# Autodesk Inventor assembly: Stock Dicoeasy Assembly-just x axis and platform
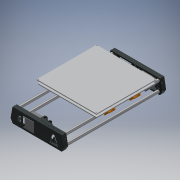
[picture p0: Inventor's stored thumbnail of the model, 180x180]
Saved by Autodesk Inventor 2017 (Build 210142000, 142)
## iProperties
Created: 2017-03-10
Part Number: Stock Dicoeasy Assembly-just x axis and platform
Document SubType Name: Assembly
Designer: gilef
Author: gilef
## Documents named in this file (14)
- C:\Users\gilef\Documents\Inventor\DiscoEasy200\Stock Dicoeasy Assembly-just x axis and platform.iam
- C:\Users\gilef\Documents\Inventor\DiscoEasy200\Original Plate Mount.ipt
- C:\Users\gilef\Documents\Inventor\DiscoEasy200\Original Rear Left Plate Mount.ipt
- C:\Users\gilef\Documents\Inventor\DiscoEasy200\Original Rear Right Plate Mount.ipt
- C:\Users\gilef\Documents\Inventor\DiscoEasy200\Converted LM8UU Linear Bearing.ipt
- C:\Users\gilef\Documents\Inventor\DiscoEasy200\Stock Build Plate.ipt
- C:\Users\gilef\Documents\Inventor\Content Center Files\R2017\en-US\AS 1427(07)\AS 1427 - M3 x 10(6) II.ipt
- C:\Users\gilef\Documents\Inventor\Content Center Files\R2017\en-US\ANSI B18.16.3M(2)\ANSI B18.16.3M - Property Class 5 and 10 - Metric M3 x 0.5 Metal Type.ipt
- C:\Users\gilef\Documents\Inventor\DiscoEasy200\Stock Front Plate.ipt
- C:\Users\gilef\Documents\Inventor\DiscoEasy200\Stock Back Plate.ipt
- C:\Users\gilef\Documents\Inventor\DiscoEasy200\Long Metal Rod.ipt
- C:\Users\gilef\Documents\Inventor\DiscoEasy200\XY Stepper Motor.ipt
- C:\Users\gilef\Documents\Inventor\DiscoEasy200\Heated Build Plate.ipt
- C:\Users\gilef\Documents\Inventor\DiscoEasy200\Plate Adapter.ipt
## Components (26 placed, 13 different names)
1. Original Plate Mount:1 — Flush:2, Mate:1, Flush:3, Mate:2, Mate:7, Mate:8, Mate:9, Mate:10, Mate:11, Insert:7, Angle:3, Insert:10, Angle:4
2. Original Rear Right Plate Mount:1 — Flush:2, Mate:1, Mate:3, Mate:4, Flush:4, Insert:9, Angle:1
3. Original Rear Left Plate Mount:1 — Flush:3, Mate:2, Mate:5, Mate:6, Flush:4, Insert:1, Insert:6, Angle:2
4. Converted LM8UU Linear Bearing:1 — Mate:7, Mate:8, Mate:15
5. Converted LM8UU Linear Bearing:2 — Mate:3, Mate:4, Mate:12
6. Converted LM8UU Linear Bearing:3 — Mate:9, Mate:10, Mate:14
7. Converted LM8UU Linear Bearing:4 — Mate:5, Mate:6, Mate:13
8. Stock Build Plate:1 — Insert:1, Mate:11, Insert:2, Insert:3, Insert:4, Insert:5, Mate:82, Angle:9, Flush:7, Flush:8, Mate:83, Mate:84, Mate:85
9. AS 1427 Z - Metric M3 x 10:1 — Insert:2
10. AS 1427 Z - Metric M3 x 10:2 — Insert:3
11. AS 1427 Z - Metric M3 x 10:3 — Insert:4
12. AS 1427 Z - Metric M3 x 10:4 — Insert:5
13. Prevailing Torque Type Hex Nut - Steel Metric Property Class 5 and 10 - Metric M3 x 0.5 Metal Type:1 — Insert:10, Angle:4
14. Prevailing Torque Type Hex Nut - Steel Metric Property Class 5 and 10 - Metric M3 x 0.5 Metal Type:2 — Insert:9, Angle:1
15. Prevailing Torque Type Hex Nut - Steel Metric Property Class 5 and 10 - Metric M3 x 0.5 Metal Type:3 — Insert:7, Angle:3
16. Prevailing Torque Type Hex Nut - Steel Metric Property Class 5 and 10 - Metric M3 x 0.5 Metal Type:4 — Insert:6, Angle:2
17. Stock Front Plate:1 — Mate:14, Mate:15, Insert:14, Insert:15, Insert:16, Insert:17, Mate:81, Angle:8, Flush:5, Flush:6
18. Stock Back Plate:1 — Mate:12, Mate:13, Insert:13, Mate:80, Tangent:1, Angle:7, Tangent:2
19. Long Metal Rod:1 — Insert:16
20. Long Metal Rod:2 — Insert:15
21. Long Metal Rod:3 — Insert:17
22. Long Metal Rod:4 — Insert:13, Insert:14
23. XY Stepper Motor:2 — Mate:80, Tangent:1, Angle:7, Tangent:2
24. XY Stepper Motor:3 — Mate:81, Angle:8, Flush:5, Flush:6
25. Heated Build Plate:1 — Mate:82, Angle:9, Flush:7, Flush:8
26. Plate Adapter:1 — Mate:83, Mate:84, Mate:85
## Relationships (51: Mate 21, Insert 14, Flush 7, Angle 7, Tangent 2)
- Flush:2: Original Plate Mount:1 ↔ Original Rear Right Plate Mount:1
- Mate:1: Original Plate Mount:1 ↔ Original Rear Right Plate Mount:1
- Flush:3: Original Plate Mount:1 ↔ Original Rear Left Plate Mount:1
- Mate:2: Original Plate Mount:1 ↔ Original Rear Left Plate Mount:1
- Mate:3: Original Rear Right Plate Mount:1 ↔ Converted LM8UU Linear Bearing:2
- Mate:4: Original Rear Right Plate Mount:1 ↔ Converted LM8UU Linear Bearing:2
- Mate:5: Original Rear Left Plate Mount:1 ↔ Converted LM8UU Linear Bearing:4
- Mate:6: Original Rear Left Plate Mount:1 ↔ Converted LM8UU Linear Bearing:4
- Mate:7: Original Plate Mount:1 ↔ Converted LM8UU Linear Bearing:1
- Mate:8: Original Plate Mount:1 ↔ Converted LM8UU Linear Bearing:1
- Mate:9: Original Plate Mount:1 ↔ Converted LM8UU Linear Bearing:3
- Mate:10: Original Plate Mount:1 ↔ Converted LM8UU Linear Bearing:3
- Flush:4: Original Rear Right Plate Mount:1 ↔ Original Rear Left Plate Mount:1
- Insert:1: Original Rear Left Plate Mount:1 ↔ Stock Build Plate:1
- Mate:11: Original Plate Mount:1 ↔ Stock Build Plate:1
- Insert:2: Stock Build Plate:1 ↔ AS 1427 Z - Metric M3 x 10:1
- Insert:3: Stock Build Plate:1 ↔ AS 1427 Z - Metric M3 x 10:2
- Insert:4: Stock Build Plate:1 ↔ AS 1427 Z - Metric M3 x 10:3
- Insert:5: Stock Build Plate:1 ↔ AS 1427 Z - Metric M3 x 10:4
- Insert:6: Original Rear Left Plate Mount:1 ↔ Prevailing Torque Type Hex Nut - Steel Metric Property Class 5 and 10 - Metric M3 x 0.5 Metal Type:4
- Insert:7: Original Plate Mount:1 ↔ Prevailing Torque Type Hex Nut - Steel Metric Property Class 5 and 10 - Metric M3 x 0.5 Metal Type:3
- Insert:9: Original Rear Right Plate Mount:1 ↔ Prevailing Torque Type Hex Nut - Steel Metric Property Class 5 and 10 - Metric M3 x 0.5 Metal Type:2
- Angle:1 (0 deg): Original Rear Right Plate Mount:1 ↔ Prevailing Torque Type Hex Nut - Steel Metric Property Class 5 and 10 - Metric M3 x 0.5 Metal Type:2
- Angle:2 (0 deg): Original Rear Left Plate Mount:1 ↔ Prevailing Torque Type Hex Nut - Steel Metric Property Class 5 and 10 - Metric M3 x 0.5 Metal Type:4
- Angle:3 (0 deg): Original Plate Mount:1 ↔ Prevailing Torque Type Hex Nut - Steel Metric Property Class 5 and 10 - Metric M3 x 0.5 Metal Type:3
- Insert:10: Original Plate Mount:1 ↔ Prevailing Torque Type Hex Nut - Steel Metric Property Class 5 and 10 - Metric M3 x 0.5 Metal Type:1
- Angle:4 (0 deg): Original Plate Mount:1 ↔ Prevailing Torque Type Hex Nut - Steel Metric Property Class 5 and 10 - Metric M3 x 0.5 Metal Type:1
- Mate:12: Converted LM8UU Linear Bearing:2 ↔ Stock Back Plate:1
- Mate:13: Converted LM8UU Linear Bearing:4 ↔ Stock Back Plate:1
- Mate:14: Converted LM8UU Linear Bearing:3 ↔ Stock Front Plate:1
- Mate:15: Converted LM8UU Linear Bearing:1 ↔ Stock Front Plate:1
- Insert:13: Stock Back Plate:1 ↔ Long Metal Rod:4
- Insert:14: Stock Front Plate:1 ↔ Long Metal Rod:4
- Insert:15: Stock Front Plate:1 ↔ Long Metal Rod:2
- Insert:16: Stock Front Plate:1 ↔ Long Metal Rod:1
- Insert:17: Stock Front Plate:1 ↔ Long Metal Rod:3
- Mate:80: Stock Back Plate:1 ↔ XY Stepper Motor:2
- Tangent:1 (0.75 mm): Stock Back Plate:1 ↔ XY Stepper Motor:2
- Angle:7 (0 deg): Stock Back Plate:1 ↔ XY Stepper Motor:2
- Tangent:2 (9 mm): Stock Back Plate:1 ↔ XY Stepper Motor:2
- Mate:81: Stock Front Plate:1 ↔ XY Stepper Motor:3
- Angle:8 (0 deg): Stock Front Plate:1 ↔ XY Stepper Motor:3
- Flush:5 (3.5 mm): Stock Front Plate:1 ↔ XY Stepper Motor:3
- Flush:6: Stock Front Plate:1 ↔ XY Stepper Motor:3
- Mate:82 (9 mm): Stock Build Plate:1 ↔ Heated Build Plate:1
- Angle:9 (0 deg): Stock Build Plate:1 ↔ Heated Build Plate:1
- Flush:7 (-1.5 mm): Stock Build Plate:1 ↔ Heated Build Plate:1
- Flush:8 (-1.5 mm): Stock Build Plate:1 ↔ Heated Build Plate:1
- Mate:83: Stock Build Plate:1 ↔ Plate Adapter:1
- Mate:84: Stock Build Plate:1 ↔ Plate Adapter:1
- Mate:85: Stock Build Plate:1 ↔ Plate Adapter:1
